# Autodesk Inventor assembly: Completa
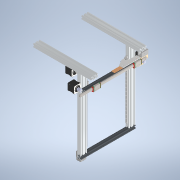
[picture p0: Inventor's stored thumbnail of the model, 180x180]
Saved by Autodesk Inventor 2021 (Build 250183000, 183)
## iProperties
Created: 2023-01-20
Part Number: Completa
Document SubType Name: Assembly
Designer: Diego.labarca
Author: Diego.labarca
## Documents named in this file (18)
- E:\Dropbox\Inventor\Impresora 3D\Arreglos Impresora\IDEX\CAD\Completa.iam
- E:\Dropbox\Inventor\Impresora 3D\Arreglos Impresora\IDEX\CAD\2040x435.ipt
- E:\Dropbox\Inventor\Impresora 3D\Arreglos Impresora\IDEX\CAD\2040x350.ipt
- E:\Dropbox\Inventor\Impresora 3D\Arreglos Impresora\IDEX\CAD\2020x330.ipt
- E:\Dropbox\Inventor\Impresora 3D\Arreglos Impresora\IDEX\CAD\MGN9x350.ipt
- E:\Dropbox\Inventor\Impresora 3D\Arreglos Impresora\IDEX\CAD\MGN9H.ipt
- E:\Dropbox\Inventor\Impresora 3D\Arreglos Impresora\IDEX\CAD\Nema17.ipt
- E:\Dropbox\Inventor\Impresora 3D\Arreglos Impresora\IDEX\CAD\Pulley GT2 20T 5ID.ipt
- E:\Dropbox\Inventor\Impresora 3D\Arreglos Impresora\IDEX\CAD\Idler GT2 20T 3ID.ipt
- E:\Dropbox\Inventor\Impresora 3D\Arreglos Impresora\IDEX\CAD\Soporte Idler Z.ipt
- E:\Dropbox\Inventor\Impresora 3D\Arreglos Impresora\IDEX\CAD\Soporte Linear Rail X.ipt
- E:\Dropbox\Inventor\Impresora 3D\Arreglos Impresora\IDEX\CAD\MGN12x350.ipt
- E:\Dropbox\Inventor\Impresora 3D\Arreglos Impresora\IDEX\CAD\MGN12H.ipt
- E:\Dropbox\Inventor\Impresora 3D\Arreglos Impresora\IDEX\CAD\Angulo 2020x450.ipt
- E:\Dropbox\Inventor\Impresora 3D\Arreglos Impresora\IDEX\CAD\Base Idler Izq.ipt
- E:\Dropbox\Inventor\Impresora 3D\Arreglos Impresora\IDEX\CAD\Soporte Motor Izq.ipt
- E:\Dropbox\Inventor\Impresora 3D\Arreglos Impresora\IDEX\CAD\MGN9H_MIR.ipt
- E:\Dropbox\Inventor\Impresora 3D\Arreglos Impresora\IDEX\CAD\MGN9x350_MIR.ipt
## Components (26 placed, 17 different names)
1. 2020x330:1 — Nivelación:4, Nivelación:5, Coincidencia:2, Coincidencia:9, Nivelación:9, Nivelación:10, Nivelación:12
2. MGN9x350:1 — Coincidencia:4, Coincidencia:5, Coincidencia:10, Coincidencia:11, Nivelación:37, Nivelación:38
3. MGN9H:1 — Coincidencia:5, Coincidencia:10, Nivelación:11, Nivelación:36
4. Nema17:1 — Coincidencia:6, Ángulo:1, Coincidencia:15
5. Pulley GT2 20T 5ID:1 — Nivelación:8, Coincidencia:15
6. Idler GT2 20T 3ID:1 — Nivelación:8, Insertar:1
7. Soporte Idler Z:1 — Coincidencia:9, Nivelación:9, Nivelación:10, Insertar:1
8. 2020x330:2 — Nivelación:12, Coincidencia:12, Coincidencia:13, Coincidencia:16, Coincidencia:17, Coincidencia:23, Coincidencia:27, Coincidencia:29, Coincidencia:30, Coincidencia:33, Coincidencia:34, Nivelación:32
9. Soporte Linear Rail X:1 — Coincidencia:13, Insertar:5
10. MGN12x350:1 — Coincidencia:16, Coincidencia:17, Coincidencia:18, Coincidencia:19, Nivelación:18, Nivelación:21, Nivelación:32, Coincidencia:40
11. MGN12H:1 — Coincidencia:18, Coincidencia:19, Nivelación:18, Nivelación:19, Nivelación:20, Coincidencia:20
12. MGN12H:2 — Nivelación:19, Nivelación:20, Coincidencia:20, Nivelación:21
13. Nema17:2 — Coincidencia:24, Coincidencia:26, Coincidencia:30, Coincidencia:35, Ángulo:3, Nivelación:33
14. Pulley GT2 20T 5ID:2 — Nivelación:27, Coincidencia:24, Nivelación:29, Nivelación:31, Ángulo:3, Coincidencia:36
15. Nema17:3 — Coincidencia:23, Coincidencia:28, Coincidencia:29
16. Pulley GT2 20T 5ID:4 — Nivelación:27, Coincidencia:27, Coincidencia:28, Coincidencia:37
17. Idler GT2 20T 3ID:2 — Nivelación:29, Nivelación:31, Coincidencia:36, Coincidencia:37
18. Angulo 2020x450:1 — Coincidencia:33, Coincidencia:34, Coincidencia:35, Nivelación:33, Nivelación:34, Coincidencia:38, Insertar:4, Coincidencia:39
19. Base Idler Izq:1 — Nivelación:34, Coincidencia:38, Insertar:4, Nivelación:35
20. Soporte Motor Izq:1 — Coincidencia:39, Nivelación:35, Coincidencia:40
21. MGN9H_MIR:1 — Coincidencia:41, Coincidencia:42, Nivelación:36, Insertar:5
22. MGN9x350_MIR:1 — Coincidencia:41, Coincidencia:42, Coincidencia:43, Nivelación:37, Nivelación:38
23. 2040x350:1 — Coincidencia:1, Nivelación:1, Nivelación:2, Coincidencia:4, Coincidencia:6, Ángulo:1
24. 2040x435:1 — Coincidencia:1, Nivelación:1, Nivelación:2, Nivelación:3, Coincidencia:11, Nivelación:11, Coincidencia:12
25. 2040x350:2
26. 2040x435:2 — Nivelación:4, Nivelación:5, Coincidencia:2, Coincidencia:26, Coincidencia:43
## Component patterns: (2 elements, first: 2040x350:1 + 2040x435:1)
## Relationships (63: Mate 34, Flush 24, Insert 3, Angle 2)
- Coincidencia:1 [Mate]: 2040x350:1 ↔ 2040x435:1
- Nivelación:1 [Flush]: 2040x350:1 ↔ 2040x435:1
- Nivelación:2 [Flush] (-65 mm): 2040x350:1 ↔ 2040x435:1
- Nivelación:3 [Flush] (-125 mm): 2040x435:1
- Nivelación:4 [Flush]: 2020x330:1 ↔ 2040x435:2
- Nivelación:5 [Flush]: 2020x330:1 ↔ 2040x435:2
- Coincidencia:2 [Mate]: 2020x330:1 ↔ 2040x435:2
- Coincidencia:4 [Mate] (50 mm): MGN9x350:1 ↔ 2040x350:1
- Coincidencia:5 [Mate]: MGN9x350:1 ↔ MGN9H:1
- Coincidencia:6 [Mate]: Nema17:1 ↔ 2040x350:1
- Nivelación:8 [Flush]: Pulley GT2 20T 5ID:1 ↔ Idler GT2 20T 3ID:1
- Ángulo:1 [Angle] (0 deg): Nema17:1 ↔ 2040x350:1
- Coincidencia:9 [Mate]: 2020x330:1 ↔ Soporte Idler Z:1
- Nivelación:9 [Flush]: 2020x330:1 ↔ Soporte Idler Z:1
- Nivelación:10 [Flush]: 2020x330:1 ↔ Soporte Idler Z:1
- Insertar:1 (1 mm): Idler GT2 20T 3ID:1 ↔ Soporte Idler Z:1
- Coincidencia:10 [Mate]: MGN9x350:1 ↔ MGN9H:1
- Coincidencia:11 [Mate]: MGN9x350:1 ↔ 2040x435:1
- Nivelación:11 [Flush]: MGN9H:1 ↔ 2040x435:1
- Nivelación:12 [Flush]: 2020x330:1 ↔ 2020x330:2
- Coincidencia:12 [Mate] (5 mm): 2020x330:2 ↔ 2040x435:1
- Coincidencia:13 [Mate]: 2020x330:2 ↔ Soporte Linear Rail X:1
- Coincidencia:15 [Mate]: Nema17:1 ↔ Pulley GT2 20T 5ID:1
- Coincidencia:16 [Mate]: 2020x330:2 ↔ MGN12x350:1
- Coincidencia:17 [Mate]: 2020x330:2 ↔ MGN12x350:1
- Coincidencia:18 [Mate]: MGN12x350:1 ↔ MGN12H:1
- Coincidencia:19 [Mate]: MGN12x350:1 ↔ MGN12H:1
- Nivelación:18 [Flush]: MGN12x350:1 ↔ MGN12H:1
- Nivelación:19 [Flush]: MGN12H:1 ↔ MGN12H:2
- Nivelación:20 [Flush]: MGN12H:1 ↔ MGN12H:2
- Coincidencia:20 [Mate]: MGN12H:1 ↔ MGN12H:2
- Nivelación:21 [Flush]: MGN12x350:1 ↔ MGN12H:2
- Coincidencia:23 [Mate] (5 mm): 2020x330:2 ↔ Nema17:3
- Nivelación:27 [Flush]: Pulley GT2 20T 5ID:2 ↔ Pulley GT2 20T 5ID:4
- Coincidencia:24 [Mate]: Nema17:2 ↔ Pulley GT2 20T 5ID:2
- Coincidencia:26 [Mate] (7 mm): Nema17:2 ↔ 2040x435:2
- Coincidencia:27 [Mate] (3.5 mm): 2020x330:2 ↔ Pulley GT2 20T 5ID:4
- Coincidencia:28 [Mate]: Nema17:3 ↔ Pulley GT2 20T 5ID:4
- Coincidencia:29 [Mate] (-2 mm): 2020x330:2 ↔ Nema17:3
- Nivelación:29 [Flush]: Pulley GT2 20T 5ID:2 ↔ Idler GT2 20T 3ID:2
- Coincidencia:30 [Mate] (-10 mm): 2020x330:2 ↔ Nema17:2
- Nivelación:31 [Flush] (45 mm): Pulley GT2 20T 5ID:2 ↔ Idler GT2 20T 3ID:2
- Coincidencia:33 [Mate]: 2020x330:2 ↔ Angulo 2020x450:1
- Coincidencia:34 [Mate]: 2020x330:2 ↔ Angulo 2020x450:1
- Nivelación:32 [Flush]: 2020x330:2 ↔ MGN12x350:1
- Coincidencia:35 [Mate]: Nema17:2 ↔ Angulo 2020x450:1
- Ángulo:3 [Angle] (0 deg): Nema17:2 ↔ Pulley GT2 20T 5ID:2
- Coincidencia:36 [Mate]: Pulley GT2 20T 5ID:2 ↔ Idler GT2 20T 3ID:2
- Coincidencia:37 [Mate]: Pulley GT2 20T 5ID:4 ↔ Idler GT2 20T 3ID:2
- Nivelación:33 [Flush]: Nema17:2 ↔ Angulo 2020x450:1
- Nivelación:34 [Flush]: Angulo 2020x450:1 ↔ Base Idler Izq:1
- Coincidencia:38 [Mate]: Angulo 2020x450:1 ↔ Base Idler Izq:1
- Insertar:4: Angulo 2020x450:1 ↔ Base Idler Izq:1
- Coincidencia:39 [Mate]: Angulo 2020x450:1 ↔ Soporte Motor Izq:1
- Nivelación:35 [Flush]: Base Idler Izq:1 ↔ Soporte Motor Izq:1
- Coincidencia:40 [Mate]: MGN12x350:1 ↔ Soporte Motor Izq:1
- Coincidencia:41 [Mate]: MGN9H_MIR:1 ↔ MGN9x350_MIR:1
- Coincidencia:42 [Mate]: MGN9H_MIR:1 ↔ MGN9x350_MIR:1
- Nivelación:36 [Flush]: MGN9H:1 ↔ MGN9H_MIR:1
- Coincidencia:43 [Mate]: MGN9x350_MIR:1 ↔ 2040x435:2
- Nivelación:37 [Flush]: MGN9x350:1 ↔ MGN9x350_MIR:1
- Nivelación:38 [Flush]: MGN9x350:1 ↔ MGN9x350_MIR:1
- Insertar:5: Soporte Linear Rail X:1 ↔ MGN9H_MIR:1
